# Autodesk Inventor assembly: Universal Shaft
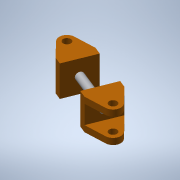
[picture p0: Inventor's stored thumbnail of the model, 180x180]
Saved by Autodesk Inventor 2022 (Build 260148000, 148)
## iProperties
Created: 2014-03-10
Part Number: Universal Shaft
Document SubType Name: Assembly
Designer: John
Author: John
## Documents named in this file (3)
- C:\Users\helfenj\Desktop\Ex_Files_Autodesk_Inventor_2022_Essential_Training\Exercise Files\12_Using constraints to position parts\12_01\Universal Shaft.iam
- C:\Users\helfenj\Desktop\Ex_Files_Autodesk_Inventor_2022_Essential_Training\Exercise Files\12_Using constraints to position parts\12_01\Joint.ipt
- C:\Users\helfenj\Desktop\Ex_Files_Autodesk_Inventor_2022_Essential_Training\Exercise Files\12_Using constraints to position parts\12_01\Connecting Rod.ipt
## Components (3 placed, 2 different names)
1. Joint:1 — Flush:3
2. Joint:2
3. Connecting Rod:1 — Flush:3
## Relationships (5: Flush 3, Mate 2)
- [Mate]: Joint:1 ↔ Joint:2
- [Flush]: Joint:1 ↔ Joint:2
- [Mate]: Joint:1 ↔ Connecting Rod:1
- [Flush]: Joint:2 ↔ Connecting Rod:1
- Flush:3: Joint:1 ↔ Connecting Rod:1
